# Autodesk Inventor assembly: 24x34 Side Rail sub
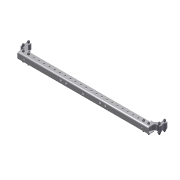
[picture p0: Inventor's stored thumbnail of the model, 180x180]
Saved by Autodesk Inventor 2013 (Build 170138000, 138)
## iProperties
Created: 2013-01-06
Part Number: 24x34 Side Rail sub
Document SubType Name: Assembly
Designer: Nemo
Author: Nemo
## Documents named in this file (4)
- H:\Nemo\Documents\Robotics\COTS Parts\Kit Frame\Components\28x28 Side Rail sub.iam
- H:\Nemo\Documents\Robotics\COTS Parts\Kit Frame\Components\CornerConnectAssyLeft.iam
- H:\Nemo\Documents\Robotics\COTS Parts\Kit Frame\Components\CornerConnectAssyRight.iam
- H:\Nemo\Documents\Robotics\COTS Parts\Kit Frame\Components\C Channel - Side 28x28.ipt
## Components (3 placed, 3 different names)
1. C Channel - Cut-01:1 — Insert:1, Mate:1, Insert:2, Mate:2
2. CornerConnectAssyLeft:1 [sub-assembly] — Insert:1, Mate:1
3. CornerConnectAssyRight:1 [sub-assembly] — Insert:2, Mate:2
## Relationships (4: Insert 2, Mate 2)
- Insert:1: C Channel - Cut-01:1 ↔ CornerConnectAssyLeft:1
- Mate:1: C Channel - Cut-01:1 ↔ CornerConnectAssyLeft:1
- Insert:2: C Channel - Cut-01:1 ↔ CornerConnectAssyRight:1
- Mate:2: C Channel - Cut-01:1 ↔ CornerConnectAssyRight:1
